# Autodesk Inventor assembly: Right
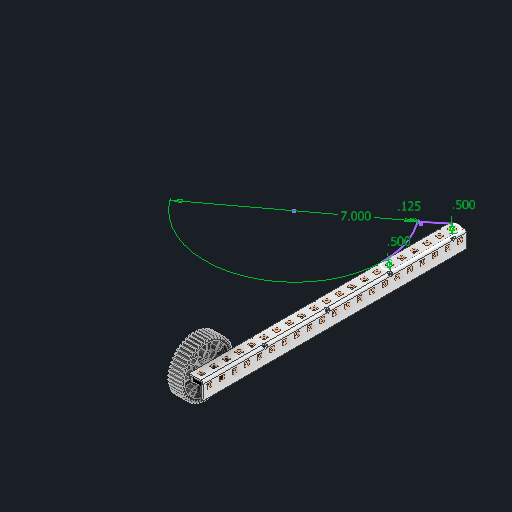
[picture p0: Inventor's stored thumbnail of the model, 512x512]
Saved by Autodesk Inventor 2025 (Build 290162000, 162)
## iProperties
Created: 2024-12-31
Part Number: Right
Document SubType Name: Assembly
Designer: Averey Ku
Author: Averey Ku
## Documents named in this file (9)
- D:\VEX\High Stakes\CAD\V4\Lady Brown\Arm\Right.iam
- D:\VEX\High Stakes\CAD\ROBOPROS-CAD-Inventor\Motion\Gears\HS Gear\HS 48T Gear, No Insert.iam
- D:\VEX\High Stakes\CAD\ROBOPROS-CAD-Inventor\Motion\Gears\HS Gear.iam
- D:\VEX\High Stakes\CAD\ROBOPROS-CAD-Inventor\Structure\C Channel\Aluminum 1x3x1 Half Thick Cut\Alu C Half Thick 1x3x1x20.ipt
- D:\VEX\High Stakes\CAD\ROBOPROS-CAD-Inventor\Structure\Standoff\Standoff .50.ipt
- D:\VEX\High Stakes\CAD\ROBOPROS-CAD-Inventor\Structure\Standoff.ipt
- D:\VEX\High Stakes\CAD\ROBOPROS-CAD-Inventor\Motion\Spacers\Washer Steel\SWasher .375 OD x .031250.ipt
- D:\VEX\High Stakes\CAD\ROBOPROS-CAD-Inventor\Motion\Spacers\Washer Steel.ipt
- D:\VEX\High Stakes\CAD\ROBOPROS-CAD-Inventor\Structure\C Channel\Aluminum 1x3x1 Half Thick Cut\Alu C Half Thick 1x3x1x21.ipt
## Components (7 placed, 5 different names)
1. HS 48T Gear, No Insert:1 [sub-assembly] — Insert:3, Insert:6
2. Alu C Half Thick 1x3x1x20:1 — Insert:4, Mate:2, Insert:7, Mate:3
3. Standoff .50:1 — Insert:2, Insert:4
4. Standoff .50:2 — Insert:5
5. SWasher .375 OD x .031250:1 — Insert:5, Insert:6, Mate:2
6. SWasher .375 OD x .031250:2 — Insert:2, Insert:3
7. Alu C Half Thick 1x3x1x21:1 — Insert:7, Mate:3
## Relationships (10: Insert 7, Mate 3)
- [Insert] (13.4938 mm): HS 48T Gear, No Insert:1 ↔ Alu C Half Thick 1x3x1x20:1
- [Mate]: HS 48T Gear, No Insert:1 ↔ Alu C Half Thick 1x3x1x20:1
- Insert:2: Standoff .50:1 ↔ SWasher .375 OD x .031250:2
- Insert:3: HS 48T Gear, No Insert:1 ↔ SWasher .375 OD x .031250:2
- Insert:4: Alu C Half Thick 1x3x1x20:1 ↔ Standoff .50:1
- Insert:5: Standoff .50:2 ↔ SWasher .375 OD x .031250:1
- Insert:6: HS 48T Gear, No Insert:1 ↔ SWasher .375 OD x .031250:1
- Mate:2: Alu C Half Thick 1x3x1x20:1 ↔ SWasher .375 OD x .031250:1
- Insert:7: Alu C Half Thick 1x3x1x20:1 ↔ Alu C Half Thick 1x3x1x21:1
- Mate:3: Alu C Half Thick 1x3x1x20:1 ↔ Alu C Half Thick 1x3x1x21:1
